# Autodesk Inventor assembly: Assembly2
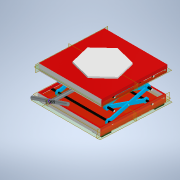
[picture p0: Inventor's stored thumbnail of the model, 180x180]
Saved by Autodesk Inventor 2020 (Build 240168000, 168)
## iProperties
Created: 2022-04-26
Part Number: Assembly2
Document SubType Name: Assembly
Designer: Manish
Author: Manish
## Documents named in this file (9)
- C:\Users\Manish\Documents\inventor\md\Project\Assembly2.iam
- C:\Users\Manish\Documents\inventor\md\Project\Part3.ipt
- C:\Users\Manish\Documents\inventor\md\Project\Part4.ipt
- C:\Users\Manish\Documents\inventor\md\Project\Part5.ipt
- C:\Users\Manish\Documents\inventor\md\Project\Part6.ipt
- C:\Users\Manish\Documents\inventor\md\Project\Part7.ipt
- C:\Users\Manish\Documents\inventor\md\Project\Part8.ipt
- C:\Users\Manish\Documents\inventor\md\Project\Part2.ipt
- C:\Users\Manish\Documents\inventor\md\Project\Part9.ipt
## Components (25 placed, 8 different names)
1. Part3:1 — Mate:3, Mate:4, Flush:1, Mate:14, Mate:17, Mate:18, Mate:21
2. Part3:2 — Mate:1, Mate:2, Mate:4, Mate:12, Mate:13, Mate:15, Mate:16, Angle:1, Mate:57
3. Part4:3 — Mate:1, Mate:2, Mate:3
4. Part3:7 — Angle:1, Mate:21, Mate:42
5. Part3:8 — Mate:19, Mate:20
6. Part4:13 — Mate:52
7. Part5:1 — Flush:1, Mate:14, Mate:20, Flush:2, Flush:3, Mate:37
8. Part5:2 — Mate:12, Mate:13, Mate:36, Mate:38
9. Part5:3 — Mate:15, Mate:16, Mate:33, Mate:45, Mate:56
10. Part5:4 — Mate:17, Mate:18, Mate:19, Mate:32, Mate:45, Flush:13, Mate:59
11. Part3:11 — Mate:33, Mate:40, Mate:42
12. Part3:12 — Mate:32, Mate:39
13. Part4:15 — Mate:53
14. Part6:1 — Flush:2, Flush:3, Mate:36, Mate:37, Mate:38, Angle:2, Angle:3, Mate:52, Mate:54, Flush:8, Flush:9
15. Part6:2 — Angle:2, Angle:3, Mate:43, Mate:44, Mate:46, Angle:4, Mate:53, Mate:54, Flush:10, Flush:11
16. Part5:5 — Mate:39, Mate:43, Flush:6, Mate:47, Mate:58, Flush:15
17. Part5:6 — Mate:40, Mate:44, Mate:50, Mate:51, Flush:13, Mate:55, Flush:15
18. Part7:1 — Mate:48, Mate:49, Flush:7, Angle:5
19. Part8:1 — Mate:46, Flush:6, Mate:47, Mate:48, Angle:5
20. Part8:2 — Mate:49, Mate:50, Angle:4, Flush:7, Mate:51
21. Part2:1 — Flush:8, Flush:9
22. Part9:1 — Flush:10, Flush:11
23. Part3:13 — Mate:55, Mate:56, Mate:57, Mate:60, Mate:61, Flush:14
24. Part3:14 — Mate:58, Mate:59, Mate:60
25. Part4:16 — Mate:61, Flush:14
## Relationships (66: Mate 49, Flush 12, Angle 5)
- Mate:1: Part3:2 ↔ Part4:3
- Mate:2: Part3:2 ↔ Part4:3
- Mate:3: Part3:1 ↔ Part4:3
- Mate:4: Part3:1 ↔ Part3:2
- [Mate]: Part3:8 ↔ Part4:13
- [Mate]: Part3:8 ↔ Part4:13
- [Mate]: Part3:7 ↔ Part4:13
- [Mate]: Part3:7 ↔ Part3:8
- Mate:12 (120 mm): Part3:2 ↔ Part5:2
- Mate:13: Part3:2 ↔ Part5:2
- Flush:1 (-120 mm): Part3:1 ↔ Part5:1
- Mate:14: Part3:1 ↔ Part5:1
- Mate:15 (120 mm): Part3:2 ↔ Part5:3
- Mate:16: Part3:2 ↔ Part5:3
- Mate:17 (120 mm): Part3:1 ↔ Part5:4
- Mate:18: Part3:1 ↔ Part5:4
- Mate:19: Part3:8 ↔ Part5:4
- Mate:20: Part3:8 ↔ Part5:1
- Angle:1 (0 deg): Part3:2 ↔ Part3:7
- Mate:21 (760 mm): Part3:1 ↔ Part3:7
- [Mate]: Part3:12 ↔ Part4:15
- [Mate]: Part3:12 ↔ Part4:15
- [Mate]: Part3:11 ↔ Part4:15
- [Mate]: Part3:11 ↔ Part3:12
- Mate:32: Part5:4 ↔ Part3:12
- Mate:33: Part5:3 ↔ Part3:11
- Flush:2: Part5:1 ↔ Part6:1
- Flush:3: Part5:1 ↔ Part6:1
- Mate:36: Part5:2 ↔ Part6:1
- Mate:37: Part5:1 ↔ Part6:1
- Mate:38 (-200 mm): Part5:2 ↔ Part6:1
- Mate:39: Part3:12 ↔ Part5:5
- Mate:40: Part3:11 ↔ Part5:6
- Mate:42: Part3:7 ↔ Part3:11
- Angle:2 (0 deg): Part6:1 ↔ Part6:2
- Angle:3 (270 deg): Part6:1 ↔ Part6:2
- Mate:43: Part6:2 ↔ Part5:5
- Mate:44 (-200 mm): Part6:2 ↔ Part5:6
- Mate:45 (600 mm): Part5:3 ↔ Part5:4
- Mate:46: Part6:2 ↔ Part8:1
- Flush:6 (-423.8 mm): Part5:5 ↔ Part8:1
- Mate:47 (-15 mm): Part5:5 ↔ Part8:1
- Mate:48: Part7:1 ↔ Part8:1
- Mate:49: Part7:1 ↔ Part8:2
- Mate:50 (-53.1 mm): Part5:6 ↔ Part8:2
- Angle:4 (0 deg): Part6:2 ↔ Part8:2
- Flush:7 (-500 mm): Part7:1 ↔ Part8:2
- Angle:5 (0 deg): Part7:1 ↔ Part8:1
- Mate:51: Part5:6 ↔ Part8:2
- Mate:52: Part4:13 ↔ Part6:1
- Mate:53: Part4:15 ↔ Part6:2
- Mate:54 (-1000 mm): Part6:1 ↔ Part6:2
- Flush:8: Part6:1 ↔ Part2:1
- Flush:9: Part6:1 ↔ Part2:1
- Flush:10: Part6:2 ↔ Part9:1
- Flush:11: Part6:2 ↔ Part9:1
- Flush:13: Part5:4 ↔ Part5:6
- Mate:55: Part5:6 ↔ Part3:13
- Mate:56: Part5:3 ↔ Part3:13
- Mate:57: Part3:2 ↔ Part3:13
- Mate:58: Part5:5 ↔ Part3:14
- Mate:59: Part5:4 ↔ Part3:14
- Mate:60: Part3:13 ↔ Part3:14
- Mate:61: Part3:13 ↔ Part4:16
- Flush:14: Part3:13 ↔ Part4:16
- Flush:15: Part5:5 ↔ Part5:6
## Named parameters: d8_d0 = 0 mm, d9_d1 = 0 mm, d10_d2 = 0 mm, d11_d3 = 0 mm, d33_d0 = 0 mm, d34_d1 = 0 mm, d35_d2 = 0 mm, d36_d3 = 0 mm
